# Autodesk Inventor assembly: GFRP_T2_03
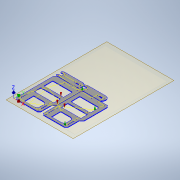
[picture p0: Inventor's stored thumbnail of the model, 180x180]
Saved by Autodesk Inventor 2020 (Build 240168000, 168)
## iProperties
Created: 2021-08-27
Part Number: GFRP_T2_03
Document SubType Name: Assembly
Designer: Masato
Author: Masato
## Documents named in this file (4)
- C:\Users\marin\Documents\0118 git clone\OpenPlatform_ver3_0\cam\GFRP_T2_03.iam
- C:\Users\marin\Documents\0118 git clone\OpenPlatform_ver3_0\cam\Disposable_Board.ipt
- C:\Users\marin\Documents\0118 git clone\OpenPlatform_ver3_0\UpperBody\Arm\ForeArm_inside_frame.ipt
- C:\Users\marin\Documents\0118 git clone\OpenPlatform_ver3_0\UpperBody\Trunk\Trunk_upper_side_frame.ipt
## Components (5 placed, 3 different names)
1. Disposable_Board:1 — メイト:2, メイト:1, フラッシュ:1, フラッシュ:2, フラッシュ:3, フラッシュ:4, メイト:5, 正接:1
2. Trunk_upper_side_frame:2 — メイト:4, フラッシュ:3, フラッシュ:4, メイト:6
3. Trunk_upper_side_frame:3
4. ForeArm_inside_frame:1 — メイト:5, 正接:1, メイト:6
5. ForeArm_inside_frame:2
## Component patterns: (2 elements, first: Trunk_upper_side_frame:2), (2 elements, first: ForeArm_inside_frame:1)
## Relationships (10: Mate 5, Flush 4, Tangent 1)
- メイト:2 [Mate]: Disposable_Board:1
- メイト:1 [Mate]: Disposable_Board:1
- フラッシュ:1 [Flush]: Disposable_Board:1
- フラッシュ:2 [Flush]: Disposable_Board:1
- メイト:4 [Mate]: Trunk_upper_side_frame:2
- フラッシュ:3 [Flush] (3 mm): Disposable_Board:1 ↔ Trunk_upper_side_frame:2
- フラッシュ:4 [Flush] (3 mm): Disposable_Board:1 ↔ Trunk_upper_side_frame:2
- メイト:5 [Mate]: Disposable_Board:1 ↔ ForeArm_inside_frame:1
- 正接:1 [Tangent] (3 mm): Disposable_Board:1 ↔ ForeArm_inside_frame:1
- メイト:6 [Mate] (2.5 mm): Trunk_upper_side_frame:2 ↔ ForeArm_inside_frame:1
